# Autodesk Inventor assembly: Reel
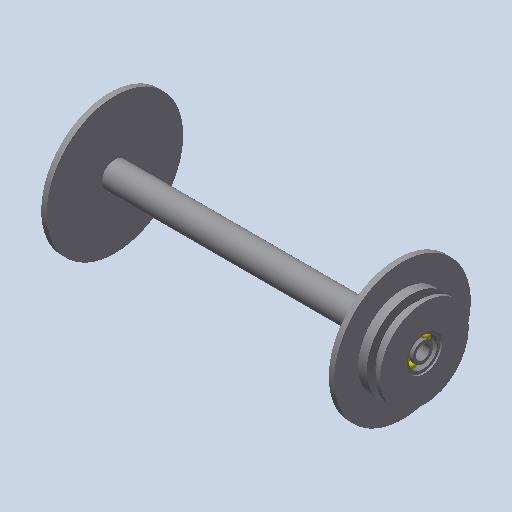
[picture p0: Inventor's stored thumbnail of the model, 512x512]
Saved by Autodesk Inventor 2022 (Build 260153000, 153)
## iProperties
Created: 2019-09-11
Part Number: Reel
Material: Genérico
Document SubType Name: Assembly
Designer: Usuario
Author: Usuario
## Documents named in this file (5)
- G:\Mi unidad\UTEC\Proyectos\Flor de Lana\Diseño 20191119\Montaje Reel.iam
- G:\Mi unidad\UTEC\Proyectos\Flor de Lana\Diseño 20191119\Torno\Centro.ipt
- G:\Mi unidad\UTEC\Proyectos\Flor de Lana\Diseño 20191119\Reel1.ipt
- G:\Mi unidad\UTEC\Proyectos\Flor de Lana\Diseño 20191119\Reel2.ipt
- G:\Mi unidad\UTEC\Proyectos\Flor de Lana\Diseño 20191119\SKF 6000\SKF_6000.iam
## Components (5 placed, 4 different names)
1. Centro:1 — Rígido:1, De rotación:1, Rigid:4
2. Reel1:1 — Rígido:1, Rigid:2
3. Reel2:1 — De rotación:1, Rigid:3
4. SKF_6000:1 [sub-assembly] — Rigid:3, Rigid:4
5. SKF_6000:2 [sub-assembly] — Rigid:2
## Relationships (5: WeldJoint 4, RevoluteJoint 1)
- Rígido:1 [WeldJoint]: Centro:1 ↔ Reel1:1
- De rotación:1 [RevoluteJoint]: Centro:1 ↔ Reel2:1
- Rigid:2 [WeldJoint]: Reel1:1 ↔ SKF_6000:2
- Rigid:3 [WeldJoint]: Reel2:1 ↔ SKF_6000:1
- Rigid:4 [WeldJoint]: Centro:1 ↔ SKF_6000:1
